# Autodesk Inventor assembly: 276-2154
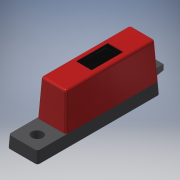
[picture p0: Inventor's stored thumbnail of the model, 180x180]
Saved by Autodesk Inventor 2019.4 (Build 234330000, 330)
## iProperties
Category: Sensors
Company: Autodesk Inc.
Created: 2012-03-26
Part Number: 276-2154
Document SubType Name: Assembly
Designer: Autodesk Inc.
Catalog Web Link: http://www.vexrobotics.com/276-2154.html
Vendor: VEX
Author: Autodesk Inc.
## Documents named in this file (6)
- D:\2019-2020TowerTakeOverCad\ncrCadLib\传感器\Line Tracker.iam
- D:\2019-2020TowerTakeOverCad\ncrCadLib\传感器\Reference Parts\Sensor Module.ipt
- D:\2019-2020TowerTakeOverCad\ncrCadLib\传感器\Reference Parts\Sensor Module Top.ipt
- D:\2019-2020TowerTakeOverCad\ncrCadLib\传感器\Reference Parts\Line Tracker Grommet.ipt
- D:\2019-2020TowerTakeOverCad\ncrCadLib\传感器\Reference Parts\Line Tracker PCB.ipt
- D:\2019-2020TowerTakeOverCad\ncrCadLib\传感器\Reference Parts\ANSI B18.6.7M - M2x0.4 x 8(5).ipt
## Components (6 placed, 5 different names)
1. Sensor Module:1 — Mate:1, Mate:2, Mate:3, Mate:4, Mate:5, Insert:1, Insert:2
2. Sensor Module Top:1 — Mate:1, Mate:4, Mate:5, Mate:6, Flush:1, Flush:2
3. Line Tracker Grommet:1 — Mate:2, Mate:3, Mate:6
4. Line Tracker PCB:1 — Flush:1, Flush:2
5. Cross Recessed Pan Head Machine Screw - Type IA - Metric M2x0.4 x 8:1 — Insert:1
6. Cross Recessed Pan Head Machine Screw - Type IA - Metric M2x0.4 x 8:2 — Insert:2
## Relationships (10: Mate 6, Flush 2, Insert 2)
- Mate:1: Sensor Module:1 ↔ Sensor Module Top:1
- Mate:2: Sensor Module:1 ↔ Line Tracker Grommet:1
- Mate:3: Sensor Module:1 ↔ Line Tracker Grommet:1
- Mate:4: Sensor Module:1 ↔ Sensor Module Top:1
- Mate:5: Sensor Module:1 ↔ Sensor Module Top:1
- Mate:6: Sensor Module Top:1 ↔ Line Tracker Grommet:1
- Flush:1: Sensor Module Top:1 ↔ Line Tracker PCB:1
- Flush:2 (-0.1524 mm): Sensor Module Top:1 ↔ Line Tracker PCB:1
- Insert:1: Sensor Module:1 ↔ Cross Recessed Pan Head Machine Screw - Type IA - Metric M2x0.4 x 8:1
- Insert:2: Sensor Module:1 ↔ Cross Recessed Pan Head Machine Screw - Type IA - Metric M2x0.4 x 8:2
